# Autodesk Inventor assembly: wire_case-1
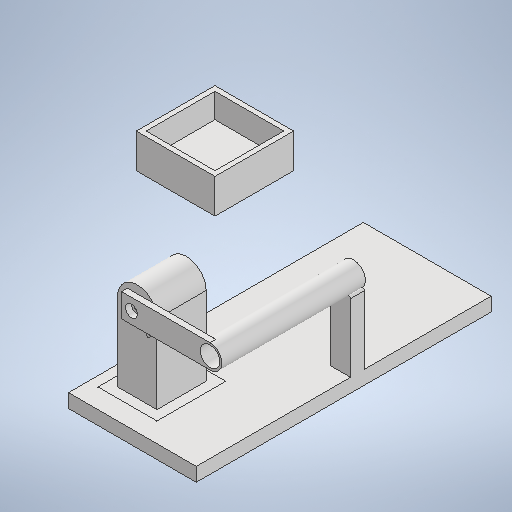
[picture p0: Inventor's stored thumbnail of the model, 512x512]
Saved by Autodesk Inventor 2025 (Build 290162000, 162)
## iProperties
Created: 2026-01-27
Part Number: wire_case-1
Document SubType Name: Assembly
Designer: mahhy
Author: mahhy
## Documents named in this file (5)
- C:\Users\mahhy\Documents\設計データ\wire_case-1\design-data\wire_case-1.iam
- C:\Users\mahhy\Documents\設計データ\wire_case-1\design-data\body-1.ipt
- C:\Users\mahhy\Documents\設計データ\wire_case-1\design-data\pole-1.ipt
- C:\Users\mahhy\Documents\設計データ\wire_case-1\design-data\body-2.ipt
- C:\Users\mahhy\Documents\設計データ\wire_case-1\design-data\box-1.ipt
## Components (4 placed, 4 different names)
1. body-1:1 — メイト:1, メイト:2, メイト:3
2. pole-1:1 — 挿入:1, 正接:1
3. body-2:1 — 挿入:1, メイト:1, メイト:2, メイト:3, 正接:1
4. box-1:1
## Relationships (5: Mate 3, Insert 1, Tangent 1)
- 挿入:1 [Insert]: pole-1:1 ↔ body-2:1
- メイト:1 [Mate]: body-1:1 ↔ body-2:1
- メイト:2 [Mate]: body-1:1 ↔ body-2:1
- メイト:3 [Mate]: body-1:1 ↔ body-2:1
- 正接:1 [Tangent]: pole-1:1 ↔ body-2:1
